# Autodesk Inventor assembly: Machine
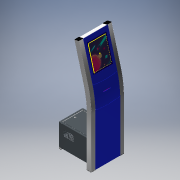
[picture p0: Inventor's stored thumbnail of the model, 180x180]
Saved by Autodesk Inventor 2016 (Build 200138000, 138)
## iProperties
Created: 2018-11-08
Part Number: Machine
Document SubType Name: Assembly
Designer: hovm
Author: hovm
## Documents named in this file (28)
- C:\Users\hovm\Desktop\DaoCM's project\Machine.iam
- C:\Users\hovm\Desktop\DaoCM's project\frame.iam
- C:\Users\hovm\Desktop\DaoCM's project\SheedSide.ipt
- C:\Users\hovm\Desktop\DaoCM's project\Sheetbottom.ipt
- C:\Users\hovm\Desktop\DaoCM's project\sheetblack.ipt
- C:\Users\hovm\Desktop\DaoCM's project\SheedSide_MIR.ipt
- C:\Users\hovm\Desktop\DaoCM's project\sheet 5.ipt
- C:\Users\hovm\Desktop\DaoCM's project\ALu.ipt
- C:\Users\hovm\Desktop\DaoCM's project\Assy Key.ipt
- C:\Users\hovm\Desktop\DaoCM's project\Screen.ipt
- C:\Users\hovm\Desktop\DaoCM's project\Part101.ipt
- C:\Users\hovm\Desktop\DaoCM's project\Part103.ipt
- C:\Users\hovm\Desktop\DaoCM's project\Part110.ipt
- C:\Users\hovm\Desktop\DaoCM's project\frame printer.iam
- C:\Users\hovm\Desktop\DaoCM's project\aluBack.ipt
- C:\Users\hovm\Desktop\DaoCM's project\Machine\Design Accelerator\Bolted Connection1.iam
- C:\Users\hovm\Desktop\DaoCM's project\79748945-9-72-7-3664\72-7-3664.iam
- C:\Users\hovm\Desktop\DaoCM's project\79748945-9-72-7-3664\72-7-3664_angle 65.iam
- C:\Users\hovm\Desktop\DaoCM's project\Part113.ipt
- C:\Users\hovm\Desktop\DaoCM's project\nút nhựa bit hộp thép 25x25.ipt
- C:\Users\hovm\Desktop\DaoCM's project\nút nhựa bịt hộp thép 60x60.ipt
- C:\Users\hovm\Desktop\DaoCM's project\Part118.ipt
- C:\Users\hovm\Desktop\DaoCM's project\Part119.ipt
- C:\Users\hovm\Desktop\DaoCM's project\Part120.ipt
- C:\Users\hovm\Desktop\DaoCM's project\Part120_MIR.ipt
- C:\Users\hovm\Desktop\DaoCM's project\Part39.ipt
- C:\Users\hovm\Desktop\DaoCM's project\Part120_MIR_MIR.ipt
- C:\Users\hovm\Desktop\DaoCM's project\Part123.ipt
## Components (48 placed, 27 different names)
1. frame:1 [sub-assembly] — Flush:1, Flush:2, Flush:3, Mate:1, Mate:2, Mate:3, Mate:4, Flush:5, Mate:5, Mate:6, Flush:6, Mate:12, Mate:14, Flush:11, Mate:29, Flush:14, Mate:30, Mate:31, Mate:32, Mate:41, Mate:42, Mate:43, Mate:44, Mate:45, Mate:46, Flush:20, Mate:47, Mate:48, Mate:49, Mate:50, Flush:21, Flush:22, Mate:51, Flush:23, Flush:24, Flush:26, Mate:54, Mate:58, Mate:59, Flush:27, Flush:28, Mate:60, Mate:61, Flush:29, Mate:62, Flush:31, Mate:64, Mate:65, Flush:32, Flush:33, Mate:73, Mate:66, Mate:67, Flush:35, Mate:68, Mate:69, Flush:37, Mate:71, Mate:72, Mate:75, Flush:40, Mate:77, Mate:78, Flush:43, Mate:79
2. SheedSide:1 — Flush:1, Flush:4, Symmetry:1
3. Sheetbottom:1 — Flush:2, Mate:76
4. sheetblack:1 — Flush:3
5. SheedSide_MIR:1 — Mate:1, Mate:2, Flush:4, Symmetry:1
6. sheet 5:1 — Mate:3, Mate:4, Flush:5, Mate:7, Mate:8
7. ALu:1 — Mate:5, Mate:6, Flush:6, Mate:9, Mate:10, Mate:11, Flush:12
8. Assy Key:1 — Mate:7, Mate:8
9. Screen:1 — Mate:9, Mate:10, Mate:11, Mate:13, Mate:17, Mate:24, Mate:55
10. Part103:1 — Mate:12, Mate:13, Flush:10, Mate:19, Mate:53
11. Part103:2 — Mate:14, Flush:10, Mate:18, Mate:52
12. Part101:3 — Mate:17, Mate:18, Mate:19, Mate:23, Flush:25
13. Part110:1 — Flush:11, Mate:21, Mate:22
14. frame printer:1 [sub-assembly] — Mate:21, Mate:22, Flush:12, Mate:33, Flush:16, Flush:17, Mate:34, Flush:18, Mate:37
15. Bolted Connection:1 [sub-assembly] — Mate:23, Mate:24
16. 72-7-3664:1 [sub-assembly] — Mate:29, Flush:14, Flush:15, Mate:31
17. 72-7-3664:2 [sub-assembly] — Mate:30, Flush:15, Mate:32
18. 72-7-3664_angle 65:1 [sub-assembly] — Mate:33, Flush:16, Flush:17, Flush:19
19. 72-7-3664_angle 65:2 [sub-assembly] — Mate:34, Flush:18, Flush:19
20. Assy Key:2 — Mate:56, Angle:1, Mate:57
21. Part113:1 — Mate:37
22. nút nhựa bit hộp thép 25x25:1 — Mate:41, Mate:42, Mate:43
23. nút nhựa bit hộp thép 25x25:2 — Mate:44, Mate:45, Mate:46
24. nút nhựa bịt hộp thép 60x60:1 — Flush:20
25. nút nhựa bịt hộp thép 60x60:2 — Mate:47, Mate:48, Mate:49
26. nút nhựa bịt hộp thép 60x60:3 — Mate:50, Flush:21, Flush:22
27. nút nhựa bịt hộp thép 60x60:4 — Mate:51, Flush:23, Flush:24
28. Part101:4 — Flush:25, Mate:52, Mate:53
29. Part118:1 — Flush:26, Mate:54, Mate:55, Mate:56, Angle:1, Mate:57, Flush:30, Mate:63, Mate:70, Flush:36, Mate:74, Flush:38
30. Part119:1 — Mate:58
31. Part120:1 — Mate:59, Flush:27, Flush:28, Mate:60
32. Part120:2 — Mate:61, Flush:29, Flush:30
33. Part120:3 — Mate:62, Flush:31, Mate:63
34. Part120:4 — Mate:64, Mate:65, Flush:32
35. aluBack:2 — Flush:33, Mate:73, Mate:66
36. Part120:7 — Mate:69, Mate:70, Flush:36
37. Part120_MIR:1
38. Part120_MIR:2
39. Part120_MIR:3 — Flush:39
40. Part39:1 — Flush:37, Mate:71, Mate:72
41. Part120_MIR:4 — Mate:74, Flush:38, Flush:39
42. Part120_MIR_MIR:1
43. Part123:1 — Mate:75, Mate:76, Flush:40, Flush:41, Flush:42
44. Part123:2 — Mate:77, Flush:41
45. Part123:3 — Flush:42, Mate:78, Flush:43, Flush:44, Flush:45
46. Part123:4 — Mate:79, Flush:44, Flush:45
47. Part120:5 — Mate:67, Flush:35, Mate:68
48. Part120:6
## Component patterns: (2 elements, first: Part120:5)
## Relationships (109: Mate 67, Flush 40, Symmetry 1, Angle 1)
- Flush:1: frame:1 ↔ SheedSide:1
- Flush:2: frame:1 ↔ Sheetbottom:1
- Flush:3: frame:1 ↔ sheetblack:1
- Mate:1: frame:1 ↔ SheedSide_MIR:1
- Mate:2: frame:1 ↔ SheedSide_MIR:1
- Flush:4: SheedSide:1 ↔ SheedSide_MIR:1
- Mate:3 (1 mm): frame:1 ↔ sheet 5:1
- Mate:4 (1 mm): frame:1 ↔ sheet 5:1
- Flush:5: frame:1 ↔ sheet 5:1
- Mate:5: frame:1 ↔ ALu:1
- Mate:6: frame:1 ↔ ALu:1
- Flush:6 (-56 mm): frame:1 ↔ ALu:1
- Mate:7: sheet 5:1 ↔ Assy Key:1
- Mate:8: sheet 5:1 ↔ Assy Key:1
- Mate:9: ALu:1 ↔ Screen:1
- Mate:10 (15 mm): ALu:1 ↔ Screen:1
- Mate:11 (15 mm): ALu:1 ↔ Screen:1
- Mate:12: frame:1 ↔ Part103:1
- Mate:13: Screen:1 ↔ Part103:1
- Mate:14: frame:1 ↔ Part103:2
- Flush:10: Part103:1 ↔ Part103:2
- Mate:17: Screen:1 ↔ Part101:3
- Mate:18: Part103:2 ↔ Part101:3
- Mate:19: Part103:1 ↔ Part101:3
- Flush:11: frame:1 ↔ Part110:1
- Mate:21: Part110:1 ↔ frame printer:1
- Mate:22: Part110:1 ↔ frame printer:1
- Flush:12 (-3.5 mm): ALu:1 ↔ frame printer:1
- Symmetry:1: SheedSide:1 ↔ SheedSide_MIR:1
- Mate:23: Part101:3 ↔ Bolted Connection:1
- Mate:24: Screen:1 ↔ Bolted Connection:1
- Mate:29: frame:1 ↔ 72-7-3664:1
- Flush:14 (-20 mm): frame:1 ↔ 72-7-3664:1
- Mate:30: frame:1 ↔ 72-7-3664:2
- Flush:15: 72-7-3664:1 ↔ 72-7-3664:2
- Mate:31 (40 mm): frame:1 ↔ 72-7-3664:1
- Mate:32 (40 mm): frame:1 ↔ 72-7-3664:2
- Mate:33: frame printer:1 ↔ 72-7-3664_angle 65:1
- Flush:16 (57.7 mm): frame printer:1 ↔ 72-7-3664_angle 65:1
- Flush:17 (10 mm): frame printer:1 ↔ 72-7-3664_angle 65:1
- Mate:34: frame printer:1 ↔ 72-7-3664_angle 65:2
- Flush:18 (10 mm): frame printer:1 ↔ 72-7-3664_angle 65:2
- Flush:19: 72-7-3664_angle 65:1 ↔ 72-7-3664_angle 65:2
- Mate:37: frame printer:1 ↔ Part113:1
- Mate:41: frame:1 ↔ nút nhựa bit hộp thép 25x25:1
- Mate:42: frame:1 ↔ nút nhựa bit hộp thép 25x25:1
- Mate:43: frame:1 ↔ nút nhựa bit hộp thép 25x25:1
- Mate:44: frame:1 ↔ nút nhựa bit hộp thép 25x25:2
- Mate:45: frame:1 ↔ nút nhựa bit hộp thép 25x25:2
- Mate:46: frame:1 ↔ nút nhựa bit hộp thép 25x25:2
- Flush:20: frame:1 ↔ nút nhựa bịt hộp thép 60x60:1
- Mate:47: frame:1 ↔ nút nhựa bịt hộp thép 60x60:2
- Mate:48: frame:1 ↔ nút nhựa bịt hộp thép 60x60:2
- Mate:49: frame:1 ↔ nút nhựa bịt hộp thép 60x60:2
- Mate:50: frame:1 ↔ nút nhựa bịt hộp thép 60x60:3
- Flush:21: frame:1 ↔ nút nhựa bịt hộp thép 60x60:3
- Flush:22: frame:1 ↔ nút nhựa bịt hộp thép 60x60:3
- Mate:51: frame:1 ↔ nút nhựa bịt hộp thép 60x60:4
- Flush:23: frame:1 ↔ nút nhựa bịt hộp thép 60x60:4
- Flush:24: frame:1 ↔ nút nhựa bịt hộp thép 60x60:4
- Flush:25: Part101:3 ↔ Part101:4
- Mate:52: Part103:2 ↔ Part101:4
- Mate:53: Part103:1 ↔ Part101:4
- Flush:26: frame:1 ↔ Part118:1
- Mate:54: frame:1 ↔ Part118:1
- Mate:55 (8 mm): Screen:1 ↔ Part118:1
- Mate:56: Assy Key:2 ↔ Part118:1
- Angle:1 (0 deg): Assy Key:2 ↔ Part118:1
- Mate:57: Assy Key:2 ↔ Part118:1
- Mate:58: frame:1 ↔ Part119:1
- Mate:59: frame:1 ↔ Part120:1
- Flush:27: frame:1 ↔ Part120:1
- Flush:28 (20 mm): frame:1 ↔ Part120:1
- Mate:60 (20 mm): frame:1 ↔ Part120:1
- Mate:61: frame:1 ↔ Part120:2
- Flush:29: frame:1 ↔ Part120:2
- Flush:30 (20 mm): Part118:1 ↔ Part120:2
- Mate:62: frame:1 ↔ Part120:3
- Flush:31: frame:1 ↔ Part120:3
- Mate:63 (20 mm): Part118:1 ↔ Part120:3
- Mate:64: frame:1 ↔ Part120:4
- Mate:65 (20 mm): frame:1 ↔ Part120:4
- Flush:32: frame:1 ↔ Part120:4
- Flush:33 (-3 mm): frame:1 ↔ aluBack:2
- Mate:73: frame:1 ↔ aluBack:2
- Mate:66 (0.5 mm): frame:1 ↔ aluBack:2
- Mate:67: frame:1 ↔ Part120:5
- Flush:35 (4 mm): frame:1 ↔ Part120:5
- Mate:68 (10 mm): frame:1 ↔ Part120:5
- Mate:69: frame:1 ↔ Part120:7
- Mate:70 (10 mm): Part118:1 ↔ Part120:7
- Flush:36 (4 mm): Part118:1 ↔ Part120:7
- Flush:37 (10 mm): frame:1 ↔ Part39:1
- Mate:71: frame:1 ↔ Part39:1
- Mate:72 (5 mm): frame:1 ↔ Part39:1
- Mate:74: Part118:1 ↔ Part120_MIR:4
- Flush:38 (60 mm): Part118:1 ↔ Part120_MIR:4
- Flush:39: Part120_MIR:3 ↔ Part120_MIR:4
- Mate:75: frame:1 ↔ Part123:1
- Mate:76 (120 mm): Sheetbottom:1 ↔ Part123:1
- Flush:40 (3 mm): frame:1 ↔ Part123:1
- Mate:77: frame:1 ↔ Part123:2
- Flush:41: Part123:1 ↔ Part123:2
- Flush:42: Part123:1 ↔ Part123:3
- Mate:78: frame:1 ↔ Part123:3
- Flush:43 (35 mm): frame:1 ↔ Part123:3
- Mate:79: frame:1 ↔ Part123:4
- Flush:44: Part123:3 ↔ Part123:4
- Flush:45: Part123:3 ↔ Part123:4
